# Autodesk Inventor assembly: BaseAssembly
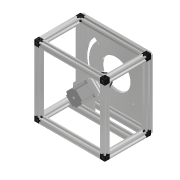
[picture p0: Inventor's stored thumbnail of the model, 180x180]
Saved by Autodesk Inventor 2020.3 (Build 243373000, 373)
## iProperties
Created: 2021-08-02
Part Number: BaseAssembly
Document SubType Name: Assembly
Designer: justi
Mass: 2934.02 g
Surface Area: 7401.15 cm^2
Volume: 1214.71 cm^3
Density: 2.41542 g/cm^3
Author: justi
## Documents named in this file (14)
- F:\UQ Engineering\2021 ~ 5th Year\Semester 2\METR4911-THESIS\FarmBot CAD\FarmBotV1\BaseAssembly_V2.iam
- F:\UQ Engineering\2021 ~ 5th Year\Semester 2\METR4911-THESIS\FarmBot CAD\FarmBotV1\LinearRail\20x20x250mm.ipt
- F:\UQ Engineering\2021 ~ 5th Year\Semester 2\METR4911-THESIS\FarmBot CAD\FarmBotV1\VSlotHardware\Cube Corner Connector.ipt
- F:\UQ Engineering\2021 ~ 5th Year\Semester 2\METR4911-THESIS\FarmBot CAD\FarmBotV1\20x20x150mm.ipt
- F:\UQ Engineering\2021 ~ 5th Year\Semester 2\METR4911-THESIS\FarmBot CAD\FarmBotV1\BaseRotation\BaseTopPlate_V2.ipt
- F:\UQ Engineering\2021 ~ 5th Year\Semester 2\METR4911-THESIS\FarmBot CAD\FarmBotV1\BasePulleyAssembly.iam
- F:\UQ Engineering\2021 ~ 5th Year\Semester 2\METR4911-THESIS\FarmBot CAD\FarmBotV1\150mm_Bearing_Plate.ipt
- F:\UQ Engineering\2021 ~ 5th Year\Semester 2\METR4911-THESIS\FarmBot CAD\FarmBotV1\GT2_TimingBelt Base.ipt
- F:\UQ Engineering\2021 ~ 5th Year\Semester 2\METR4911-THESIS\FarmBot CAD\FarmBotV1\BaseAssembly_V2\AIP\FEA\drtoetzj4.fins
- F:\UQ Engineering\2021 ~ 5th Year\Semester 2\METR4911-THESIS\FarmBot CAD\FarmBotV1\BaseAssembly_V2\AIP\FEA\drtoetzk0.fsat
- F:\UQ Engineering\2021 ~ 5th Year\Semester 2\METR4911-THESIS\FarmBot CAD\FarmBotV1\BaseAssembly_V2\AIP\FEA\drtoetzkw.ftes
- F:\UQ Engineering\2021 ~ 5th Year\Semester 2\METR4911-THESIS\FarmBot CAD\FarmBotV1\BaseAssembly_V2\AIP\FEA\drtoetzls.fwiz
- F:\UQ Engineering\2021 ~ 5th Year\Semester 2\METR4911-THESIS\FarmBot CAD\FarmBotV1\BaseAssembly_V2\AIP\FEA\drtoeu08w.fmsh
- F:\UQ Engineering\2021 ~ 5th Year\Semester 2\METR4911-THESIS\FarmBot CAD\FarmBotV1\BaseAssembly_V2\AIP\FEA\drtoeu09s.fres
## Components (25 placed, 7 different names)
1. 20x20x250mm:2 — Mate:47, Flush:1, Flush:2, Mate:50, Flush:7, Flush:8, Flush:41
2. Cube Corner Connector:3 — Mate:47, Flush:1, Flush:2, Flush:15, Mate:54, Flush:16, Flush:17
3. 20x20x250mm:3 — Flush:13, Flush:14
4. Cube Corner Connector:4 — Flush:9, Mate:52, Flush:10, Mate:56, Flush:20, Flush:21
5. 20x20x250mm:4 — Flush:9, Mate:52, Flush:10
6. Cube Corner Connector:5 — Mate:50, Flush:7, Flush:8, Mate:55, Flush:18, Flush:19
7. 20x20x250mm:5 — Flush:15, Flush:45
8. Cube Corner Connector:6 — Flush:13, Flush:14, Mate:57, Flush:22, Flush:23
9. 20x20x150mm:1 — Mate:54, Flush:16, Flush:17, Mate:64, Flush:39, Flush:40, Flush:42
10. 20x20x150mm:2 — Mate:55, Flush:18, Flush:19
11. 20x20x150mm:3 — Mate:56, Flush:20, Flush:21
12. 20x20x150mm:4 — Mate:57, Flush:22, Flush:23, Mate:70, Mate:71, Flush:46, Mate:73
13. 20x20x250mm:6
14. Cube Corner Connector:7 — Mate:64, Flush:39, Flush:40
15. 20x20x250mm:7
16. Cube Corner Connector:8
17. 20x20x250mm:8
18. Cube Corner Connector:9
19. 20x20x250mm:9
20. Cube Corner Connector:10 — Mate:69
21. BaseTopPlate_V2:1 — Flush:41, Flush:42, Flush:43, Flush:44, Mate:69, Mate:74, Mate:75, Mate:76
22. 20x20x250mm:10 — Mate:70, Mate:71, Flush:45, Mate:72
23. BasePulleyAssembly:1 [sub-assembly] — Flush:46, Mate:72, Mate:73, Mate:77, Mate:78, Mate:79
24. 150mm_Bearing_Plate:1 — Mate:74, Mate:75, Mate:76
25. GT2_TimingBelt Base:1 — Mate:77, Mate:78, Mate:79
## Relationships (74: Flush 46, Mate 28)
- Mate:47: 20x20x250mm:2 ↔ Cube Corner Connector:3
- Flush:1: 20x20x250mm:2 ↔ Cube Corner Connector:3
- Flush:2: 20x20x250mm:2 ↔ Cube Corner Connector:3
- [Mate]: 20x20x250mm:3 ↔ Cube Corner Connector:4
- [Flush]: 20x20x250mm:3 ↔ Cube Corner Connector:4
- [Flush]: 20x20x250mm:3 ↔ Cube Corner Connector:4
- [Mate]: 20x20x250mm:4 ↔ Cube Corner Connector:5
- [Flush]: 20x20x250mm:4 ↔ Cube Corner Connector:5
- [Flush]: 20x20x250mm:4 ↔ Cube Corner Connector:5
- Mate:50: 20x20x250mm:2 ↔ Cube Corner Connector:5
- Flush:7: 20x20x250mm:2 ↔ Cube Corner Connector:5
- Flush:8: 20x20x250mm:2 ↔ Cube Corner Connector:5
- Flush:9: Cube Corner Connector:4 ↔ 20x20x250mm:4
- Mate:52: Cube Corner Connector:4 ↔ 20x20x250mm:4
- Flush:10: Cube Corner Connector:4 ↔ 20x20x250mm:4
- [Mate]: 20x20x250mm:5 ↔ Cube Corner Connector:6
- [Flush]: 20x20x250mm:5 ↔ Cube Corner Connector:6
- [Flush]: 20x20x250mm:5 ↔ Cube Corner Connector:6
- Flush:13: 20x20x250mm:3 ↔ Cube Corner Connector:6
- Flush:14: 20x20x250mm:3 ↔ Cube Corner Connector:6
- Flush:15: Cube Corner Connector:3 ↔ 20x20x250mm:5
- Mate:54: Cube Corner Connector:3 ↔ 20x20x150mm:1
- Flush:16: Cube Corner Connector:3 ↔ 20x20x150mm:1
- Flush:17: Cube Corner Connector:3 ↔ 20x20x150mm:1
- Mate:55: Cube Corner Connector:5 ↔ 20x20x150mm:2
- Flush:18: Cube Corner Connector:5 ↔ 20x20x150mm:2
- Flush:19: Cube Corner Connector:5 ↔ 20x20x150mm:2
- Mate:56: Cube Corner Connector:4 ↔ 20x20x150mm:3
- Flush:20: Cube Corner Connector:4 ↔ 20x20x150mm:3
- Flush:21: Cube Corner Connector:4 ↔ 20x20x150mm:3
- Mate:57: Cube Corner Connector:6 ↔ 20x20x150mm:4
- Flush:22: Cube Corner Connector:6 ↔ 20x20x150mm:4
- Flush:23: Cube Corner Connector:6 ↔ 20x20x150mm:4
- [Mate]: 20x20x250mm:6 ↔ Cube Corner Connector:7
- [Flush]: 20x20x250mm:6 ↔ Cube Corner Connector:7
- [Flush]: 20x20x250mm:6 ↔ Cube Corner Connector:7
- [Mate]: 20x20x250mm:7 ↔ Cube Corner Connector:8
- [Flush]: 20x20x250mm:7 ↔ Cube Corner Connector:8
- [Flush]: 20x20x250mm:7 ↔ Cube Corner Connector:8
- [Mate]: 20x20x250mm:8 ↔ Cube Corner Connector:9
- [Flush]: 20x20x250mm:8 ↔ Cube Corner Connector:9
- [Flush]: 20x20x250mm:8 ↔ Cube Corner Connector:9
- [Mate]: 20x20x250mm:6 ↔ Cube Corner Connector:9
- [Flush]: 20x20x250mm:6 ↔ Cube Corner Connector:9
- [Flush]: 20x20x250mm:6 ↔ Cube Corner Connector:9
- [Flush]: Cube Corner Connector:8 ↔ 20x20x250mm:8
- [Mate]: Cube Corner Connector:8 ↔ 20x20x250mm:8
- [Flush]: Cube Corner Connector:8 ↔ 20x20x250mm:8
- [Mate]: 20x20x250mm:9 ↔ Cube Corner Connector:10
- [Flush]: 20x20x250mm:9 ↔ Cube Corner Connector:10
- [Flush]: 20x20x250mm:9 ↔ Cube Corner Connector:10
- [Flush]: 20x20x250mm:7 ↔ Cube Corner Connector:10
- [Flush]: 20x20x250mm:7 ↔ Cube Corner Connector:10
- [Flush]: Cube Corner Connector:7 ↔ 20x20x250mm:9
- Mate:64: 20x20x150mm:1 ↔ Cube Corner Connector:7
- Flush:39: 20x20x150mm:1 ↔ Cube Corner Connector:7
- Flush:40: 20x20x150mm:1 ↔ Cube Corner Connector:7
- Flush:41: 20x20x250mm:2 ↔ BaseTopPlate_V2:1
- Flush:42: 20x20x150mm:1 ↔ BaseTopPlate_V2:1
- Flush:43 (-145 mm): BaseTopPlate_V2:1
- Flush:44 (-145 mm): BaseTopPlate_V2:1
- Mate:69: Cube Corner Connector:10 ↔ BaseTopPlate_V2:1
- Mate:70: 20x20x150mm:4 ↔ 20x20x250mm:10
- Mate:71: 20x20x150mm:4 ↔ 20x20x250mm:10
- Flush:45 (-119.3 mm): 20x20x250mm:5 ↔ 20x20x250mm:10
- Flush:46: 20x20x150mm:4 ↔ BasePulleyAssembly:1
- Mate:72: 20x20x250mm:10 ↔ BasePulleyAssembly:1
- Mate:73: 20x20x150mm:4 ↔ BasePulleyAssembly:1
- Mate:74: BaseTopPlate_V2:1 ↔ 150mm_Bearing_Plate:1
- Mate:75: BaseTopPlate_V2:1 ↔ 150mm_Bearing_Plate:1
- Mate:76: BaseTopPlate_V2:1 ↔ 150mm_Bearing_Plate:1
- Mate:77: BasePulleyAssembly:1 ↔ GT2_TimingBelt Base:1
- Mate:78: BasePulleyAssembly:1 ↔ GT2_TimingBelt Base:1
- Mate:79: BasePulleyAssembly:1 ↔ GT2_TimingBelt Base:1
## Named parameters: d97_d94 = 0 mm, d98_d95 = 0 mm, d99_d96 = 0 mm, d100_d94 = 0 mm, d101_d95 = 0 mm, d102_d96 = 0 mm, d110_d94 = 0 mm, d111_d95 = 0 mm, d112_d96 = 0 mm, d128_d106 = 0 mm, d129_d108 = 0 mm, d130_d109 = 0 mm, d131_d110_d94 = 0 mm, d132_d111_d95 = 0 mm, d133_d112_d96 = 0 mm, d134_d113 = 0 mm, d135_d114 = 0 mm, d136_d115 = 0 mm, d137_d94 = 0 mm, d138_d95 = 0 mm, d139_d96 = 0 mm, d140_d97_d94 = 0 mm, d141_d98_d95 = 0 mm, d142_d99_d96 = 0 mm, d143_d100_d94 = 0 mm, d144_d101_d95 = 0 mm, d145_d102_d96 = 0 mm, d146_d103 = 0 mm, d147_d104 = 0 mm, d148_d105 = 0 mm, sa_0 = 49050, sa_1 = 981
note: some values were not read from the file. Shown as the stored number, unit unknown: "sa_0", "sa_1".
